# Autodesk Inventor assembly: Actuator 1.6
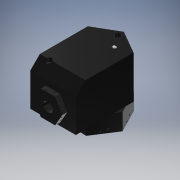
[picture p0: Inventor's stored thumbnail of the model, 180x180]
Saved by Autodesk Inventor 2017 (Build 210142000, 142)
## iProperties
Created: 2019-09-19
Part Number: Actuator 1.6
Document SubType Name: Assembly
Designer: Dell
Author: Dell
## Documents named in this file (16)
- C:\Users\Dell\Documents\GitHub\tr2\Actuator 1.6\Actuator 1.6.iam
- C:\Users\Dell\Documents\GitHub\tr2\Actuator 1.6\AC01.ipt
- C:\Users\Dell\Documents\GitHub\tr2\Actuator 1.6\AC02.ipt
- C:\Users\Dell\Documents\GitHub\tr2\Actuator 1.6\AC03.ipt
- C:\Users\Dell\Documents\GitHub\tr2\Actuator 1.6\AC05.ipt
- C:\Users\Dell\Documents\GitHub\tr2\Actuator 1.6\Slewing.iam
- C:\Users\Dell\Documents\GitHub\tr2\Actuator 1.6\TSINY TS-42GZ495.ipt
- C:\Users\Dell\Documents\GitHub\tr2\Actuator 1.6\Slip Ring.ipt
- C:\Users\Dell\Documents\GitHub\tr2\Actuator 1.6\8mm Mounting Hub.ipt
- C:\Users\Dell\Documents\GitHub\tr2\Actuator 1.6\Actuator 1.6\Design Accelerator\Spur Gears1.iam
- C:\Users\Dell\Documents\GitHub\tr2\Actuator 1.6\AEAT-6012.ipt
- C:\Users\Dell\Documents\GitHub\tr2\Actuator 1.6\Actuator 1.6\Design Accelerator\Spur Gears2.iam
- C:\Users\Dell\Documents\GitHub\tr2\Actuator 1.6\AC06.ipt
- C:\Users\Dell\Documents\GitHub\tr2\Actuator 1.6\AC07.ipt
- C:\Users\Dell\Documents\GitHub\tr2\Actuator 1.6\Series Elastic Gearbox 1.2\Series Elastic Gearbox 1.2.iam
- C:\Users\Dell\Documents\GitHub\tr2\Actuator 1.6\AC08.ipt
## Components (17 placed, 14 different names)
1. AC01:1 — Mate:3, Mate:4, Mate:5, Mate:9, Mate:11, Mate:19, Flush:1
2. AC02:1 — Mate:9, Mate:11, Mate:14, Mate:15, Mate:16, Mate:17, Mate:18, Mate:19, Mate:27, Mate:70, Mate:71, Mate:72, Mate:76, Mate:77, Mate:78, Mate:113
3. AC03:1 — Mate:16, Mate:17, Mate:18
4. AC05:1 — Mate:6, Mate:7, Mate:8, Mate:23, Mate:24, Mate:25, Mate:90, Mate:91, Mate:92
5. Slewing:1 [sub-assembly] — Mate:3, Mate:4, Mate:5, Mate:6, Mate:7, Mate:8
6. TSINY TS-42GZ495:1 — Mate:14, Mate:15, Mate:26, Mate:27, Mate:28
7. Slip Ring:2 — Mate:23, Mate:24, Mate:25
8. 8mm Mounting Hub:1 — Mate:26, Mate:28, Mate:102, Mate:103, Mate:115
9. Spur Gears:1 [sub-assembly] — Rotation:1, Mate:93, Mate:94, Mate:95, Mate:104, Mate:115, Mate:116, Mate:117, Mate:118, Mate:119
10. AEAT-6012:1 — Mate:79, Mate:80, Mate:88
11. AEAT-6012:2 — Mate:73, Mate:74, Mate:89
12. Spur Gears:2 [sub-assembly] — Mate:75, Mate:76, Mate:79, Mate:96, Mate:97, Mate:111, Mate:112, Mate:113, Mate:114
13. AC06:1 — Flush:1, Rotation:1, Mate:72, Mate:73
14. AC07:1 — Mate:70, Mate:71, Mate:74, Mate:89
15. AC07:2 — Mate:75, Mate:77, Mate:78, Mate:80, Mate:88
16. AC08:1 — Mate:102, Mate:103, Mate:104, Mate:116, Mate:119
17. Series Elastic Gearbox 1.2:1 [sub-assembly] — Mate:90, Mate:91, Mate:92, Mate:93, Mate:94, Mate:95, Mate:96, Mate:97, Mate:111, Mate:112, Mate:114, Mate:117, Mate:118
## Relationships (55: Mate 53, Flush 1, RelateRotation 1)
- Mate:3: AC01:1 ↔ Slewing:1
- Mate:4: AC01:1 ↔ Slewing:1
- Mate:5: AC01:1 ↔ Slewing:1
- Mate:6: AC05:1 ↔ Slewing:1
- Mate:7: AC05:1 ↔ Slewing:1
- Mate:8: AC05:1 ↔ Slewing:1
- Mate:9: AC01:1 ↔ AC02:1
- Mate:11: AC01:1 ↔ AC02:1
- Mate:14: AC02:1 ↔ TSINY TS-42GZ495:1
- Mate:15: AC02:1 ↔ TSINY TS-42GZ495:1
- Mate:16: AC02:1 ↔ AC03:1
- Mate:17: AC02:1 ↔ AC03:1
- Mate:18: AC02:1 ↔ AC03:1
- Mate:19: AC01:1 ↔ AC02:1
- Mate:23: AC05:1 ↔ Slip Ring:2
- Mate:24 (5 mm): AC05:1 ↔ Slip Ring:2
- Mate:25: AC05:1 ↔ Slip Ring:2
- Mate:26: TSINY TS-42GZ495:1 ↔ 8mm Mounting Hub:1
- Mate:27: AC02:1 ↔ TSINY TS-42GZ495:1
- Mate:28 (3 mm): TSINY TS-42GZ495:1 ↔ 8mm Mounting Hub:1
- Flush:1: AC01:1 ↔ AC06:1
- Rotation:1 [RelateRotation] (0.7 ul): Spur Gears:1 ↔ AC06:1
- Mate:70: AC02:1 ↔ AC07:1
- Mate:71: AC02:1 ↔ AC07:1
- Mate:72: AC02:1 ↔ AC06:1
- Mate:73: AEAT-6012:2 ↔ AC06:1
- Mate:74: AEAT-6012:2 ↔ AC07:1
- Mate:75: Spur Gears:2 ↔ AC07:2
- Mate:76: AC02:1 ↔ Spur Gears:2
- Mate:77: AC02:1 ↔ AC07:2
- Mate:78: AC02:1 ↔ AC07:2
- Mate:79: AEAT-6012:1 ↔ Spur Gears:2
- Mate:80: AEAT-6012:1 ↔ AC07:2
- Mate:88: AEAT-6012:1 ↔ AC07:2
- Mate:89: AEAT-6012:2 ↔ AC07:1
- Mate:90: AC05:1 ↔ Series Elastic Gearbox 1.2:1
- Mate:91: AC05:1 ↔ Series Elastic Gearbox 1.2:1
- Mate:92: AC05:1 ↔ Series Elastic Gearbox 1.2:1
- Mate:93: Spur Gears:1 ↔ Series Elastic Gearbox 1.2:1
- Mate:94: Spur Gears:1 ↔ Series Elastic Gearbox 1.2:1
- Mate:95: Spur Gears:1 ↔ Series Elastic Gearbox 1.2:1
- Mate:96: Spur Gears:2 ↔ Series Elastic Gearbox 1.2:1
- Mate:97: Spur Gears:2 ↔ Series Elastic Gearbox 1.2:1
- Mate:102: 8mm Mounting Hub:1 ↔ AC08:1
- Mate:103: 8mm Mounting Hub:1 ↔ AC08:1
- Mate:104: Spur Gears:1 ↔ AC08:1
- Mate:111: Spur Gears:2 ↔ Series Elastic Gearbox 1.2:1
- Mate:112: Spur Gears:2 ↔ Series Elastic Gearbox 1.2:1
- Mate:113: AC02:1 ↔ Spur Gears:2
- Mate:114: Spur Gears:2 ↔ Series Elastic Gearbox 1.2:1
- Mate:115: 8mm Mounting Hub:1 ↔ Spur Gears:1
- Mate:116: Spur Gears:1 ↔ AC08:1
- Mate:117: Spur Gears:1 ↔ Series Elastic Gearbox 1.2:1
- Mate:118: Spur Gears:1 ↔ Series Elastic Gearbox 1.2:1
- Mate:119: Spur Gears:1 ↔ AC08:1
